# Autodesk Inventor assembly: FullArm
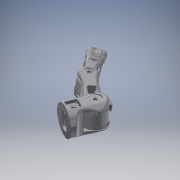
[picture p0: Inventor's stored thumbnail of the model, 180x180]
Saved by Autodesk Inventor 2019 (Build 230136000, 136)
## iProperties
Created: 2020-03-22
Part Number: FullArm
Document SubType Name: Assembly
Designer: james
Author: james
## Documents named in this file (5)
- F:\JimsRobot\FIRSTRobots\Design\RBX1-REMIX\FullArm.iam
- F:\JimsRobot\FIRSTRobots\Design\RBX1-REMIX\forearm\forearm.iam
- F:\JimsRobot\FIRSTRobots\Design\RBX1-REMIX\arm\arm.iam
- F:\JimsRobot\FIRSTRobots\Design\RBX1-REMIX\shoulder\shoulder.iam
- F:\JimsRobot\FIRSTRobots\Design\RBX1-REMIX\wrist\wrist.iam
## Components (4 placed, 4 different names)
1. forearm:1 [sub-assembly] — Mate:1, Mate:2, Mate:5, Mate:6
2. arm:1 [sub-assembly] — Mate:1, Mate:2, Mate:3, Mate:7
3. shoulder:1 [sub-assembly] — Mate:3, Mate:7
4. wrist:1 [sub-assembly] — Mate:5, Mate:6
## Relationships (6: Mate 6)
- Mate:1: forearm:1 ↔ arm:1
- Mate:2: forearm:1 ↔ arm:1
- Mate:3: arm:1 ↔ shoulder:1
- Mate:5: forearm:1 ↔ wrist:1
- Mate:6: forearm:1 ↔ wrist:1
- Mate:7: arm:1 ↔ shoulder:1
